# Autodesk Inventor assembly: WheelAssembly3.0
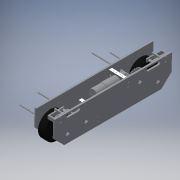
[picture p0: Inventor's stored thumbnail of the model, 180x180]
Saved by Autodesk Inventor 2017 (Build 210142000, 142)
## iProperties
Created: 2017-07-22
Part Number: WheelAssembly3.0
Document SubType Name: Assembly
Designer: User
Author: User
## Documents named in this file (15)
- C:\Robotics\CAD\2017-18_CAD\Miscellaneous\WheelAssembly3.0.iam
- C:\Robotics\CAD\2016-17_CAD\DriveTrain\DriveTrainPlateInside3.0.ipt
- C:\Robotics\CAD\COTSParts\Motors\Andymark 2964  NeveRest 40 Motor.ipt
- C:\Robotics\CAD\COTSParts\Tetrix\tetrix-motor-mounts-1.snapshot.1\Tetrex 2pc motor mount.ipt
- C:\Robotics\CAD\COTSParts\Actobotics\615 parts\615398.25inBoreBeveledGears.ipt
- C:\Robotics\CAD\2016-17_CAD\Custom COTS\4inax.ipt
- C:\Robotics\CAD\COTSParts\Actobotics\615 parts\615106Sprocket.5inBore.25inPitch24Teeth.ipt
- C:\Robotics\CAD\COTSParts\Actobotics\545 parts\545556SetScrewHub.77inPattern.ipt
- C:\Robotics\CAD\COTSParts\Actobotics\615 parts\615114Sprocket.5inBore.25inPitch32Teeth.ipt
- C:\Robotics\CAD\2016-17_CAD\DriveTrain\Tensioner.iam
- C:\Robotics\CAD\COTSParts\Actobotics\545 parts\545456PatternAdapter.77in.625in.ipt
- C:\Robotics\CAD\COTSParts\Wheels\4in Wheel Intergreated Hub 8mm Rev2.ipt
- C:\Robotics\CAD\2016-17_CAD\DriveTrain\MotorFixedPositionMount.ipt
- C:\Robotics\CAD\COTSParts\Actobotics\Thrust Bearings\6655K13.ipt
- C:\Robotics\CAD\2016-17_CAD\DriveTrain\DriveTrainPlateOutside3.0.ipt
## Components (36 placed, 14 different names)
1. DriveTrainPlateInside3.0:1 — Flush:3, Flush:4, Mate:2, Flush:5, Mate:3, Flush:6, Angle:1, Insert:7, Insert:8, Angle:2, Insert:9, Insert:10, Insert:16, Insert:17, Flush:17, Flush:18, Mate:21, Flush:19, Mate:22, Flush:20
2. Andymark 2964  NeveRest 40 Motor:1 — Insert:3, Insert:6, Angle:2
3. Andymark 2964  NeveRest 40 Motor:2 — Insert:4, Insert:5, Angle:1
4. Tetrex 2pc motor mount:1 — Insert:3, Flush:3, Mate:3, Flush:6, Mate:27, Insert:48, Angle:3
5. Tetrex 2pc motor mount:2 — Insert:4, Flush:4, Mate:2, Flush:5, Insert:30, Angle:4
6. 615398.25inBoreBeveledGears:1 — Insert:5, Insert:44
7. 615398.25inBoreBeveledGears:2 — Insert:6, Insert:47
8. 615398.25inBoreBeveledGears:3 — Insert:7, Insert:36
9. 615398.25inBoreBeveledGears:4 — Insert:8, Insert:38
10. 4inax:1 — Insert:9, Mate:18
11. 4inax:2 — Insert:10, Mate:19, Mate:23, Mate:26
12. 615106Sprocket.5inBore.25inPitch24Teeth:2 — Insert:26, Flush:21
13. 4inax:3 — Insert:16
14. 4inax:4 — Insert:17, Mate:14, Mate:25
15. 545556SetScrewHub.77inPattern:3 — Insert:26, Mate:14
16. 615114Sprocket.5inBore.25inPitch32Teeth:2 — Insert:37, Flush:21
17. 545556SetScrewHub.77inPattern:4 — Insert:36, Insert:37, Insert:43
18. Tensioner:1 [sub-assembly] — Flush:17, Flush:18, Mate:21
19. 545556SetScrewHub.77inPattern:5 — Mate:23, Insert:40
20. 545456PatternAdapter.77in.625in:1 — Insert:40, Insert:41
21. 4in Wheel Intergreated Hub 8mm Rev2:1 — Insert:41, Insert:50
22. Tensioner:2 [sub-assembly] — Flush:19, Mate:22, Flush:20
23. 545556SetScrewHub.77inPattern:6 — Insert:27
24. 545456PatternAdapter.77in.625in:2 — Insert:27, Insert:28
25. 4in Wheel Intergreated Hub 8mm Rev2:2 — Insert:28, Insert:49
26. MotorFixedPositionMount:1 — Insert:30, Angle:4
27. MotorFixedPositionMount:2 — Insert:48, Angle:3
28. 545556SetScrewHub.77inPattern:7 — Mate:18, Insert:38, Insert:39, Insert:42
29. 545556SetScrewHub.77inPattern:8 — Insert:35, Mate:19
30. 615114Sprocket.5inBore.25inPitch32Teeth:3 — Insert:39, Flush:22
31. 615106Sprocket.5inBore.25inPitch24Teeth:3 — Insert:35, Flush:22
32. 6655K13:1 — Insert:42
33. 6655K13:2 — Insert:43
34. 6655K13:3 — Insert:44
35. DriveTrainPlateOutside3.0:1 — Mate:25, Mate:26, Mate:27, Insert:49, Insert:50
36. 6655K13:4 — Insert:47
## Relationships (53: Insert 28, Mate 11, Flush 10, Angle 4)
- Insert:3: Andymark 2964  NeveRest 40 Motor:1 ↔ Tetrex 2pc motor mount:1
- Insert:4: Andymark 2964  NeveRest 40 Motor:2 ↔ Tetrex 2pc motor mount:2
- Flush:3 (159.5374 mm): DriveTrainPlateInside3.0:1 ↔ Tetrex 2pc motor mount:1
- Flush:4 (159.5374 mm): DriveTrainPlateInside3.0:1 ↔ Tetrex 2pc motor mount:2
- Insert:5: Andymark 2964  NeveRest 40 Motor:2 ↔ 615398.25inBoreBeveledGears:1
- Mate:2: DriveTrainPlateInside3.0:1 ↔ Tetrex 2pc motor mount:2
- Flush:5 (7.3152 mm): DriveTrainPlateInside3.0:1 ↔ Tetrex 2pc motor mount:2
- Mate:3: DriveTrainPlateInside3.0:1 ↔ Tetrex 2pc motor mount:1
- Flush:6 (-20.3454 mm): DriveTrainPlateInside3.0:1 ↔ Tetrex 2pc motor mount:1
- Angle:1 (0 deg): DriveTrainPlateInside3.0:1 ↔ Andymark 2964  NeveRest 40 Motor:2
- Insert:6: Andymark 2964  NeveRest 40 Motor:1 ↔ 615398.25inBoreBeveledGears:2
- Insert:7 (25.4508 mm): DriveTrainPlateInside3.0:1 ↔ 615398.25inBoreBeveledGears:3
- Insert:8 (25.4508 mm): DriveTrainPlateInside3.0:1 ↔ 615398.25inBoreBeveledGears:4
- Angle:2 (180 deg): DriveTrainPlateInside3.0:1 ↔ Andymark 2964  NeveRest 40 Motor:1
- Insert:9 (-6.35 mm): DriveTrainPlateInside3.0:1 ↔ 4inax:1
- Insert:10 (-6.35 mm): DriveTrainPlateInside3.0:1 ↔ 4inax:2
- Insert:16 (-6.35 mm): DriveTrainPlateInside3.0:1 ↔ 4inax:3
- Insert:17 (-6.35 mm): DriveTrainPlateInside3.0:1 ↔ 4inax:4
- Insert:26: 615106Sprocket.5inBore.25inPitch24Teeth:2 ↔ 545556SetScrewHub.77inPattern:3
- Mate:14: 4inax:4 ↔ 545556SetScrewHub.77inPattern:3
- Insert:27: 545556SetScrewHub.77inPattern:6 ↔ 545456PatternAdapter.77in.625in:2
- Insert:28: 545456PatternAdapter.77in.625in:2 ↔ 4in Wheel Intergreated Hub 8mm Rev2:2
- Insert:30: Tetrex 2pc motor mount:2 ↔ MotorFixedPositionMount:1
- Insert:35: 545556SetScrewHub.77inPattern:8 ↔ 615106Sprocket.5inBore.25inPitch24Teeth:3
- Mate:18: 4inax:1 ↔ 545556SetScrewHub.77inPattern:7
- Mate:19: 4inax:2 ↔ 545556SetScrewHub.77inPattern:8
- Flush:17: DriveTrainPlateInside3.0:1 ↔ Tensioner:1
- Flush:18 (34.925 mm): DriveTrainPlateInside3.0:1 ↔ Tensioner:1
- Mate:21: DriveTrainPlateInside3.0:1 ↔ Tensioner:1
- Flush:19: DriveTrainPlateInside3.0:1 ↔ Tensioner:2
- Mate:22: DriveTrainPlateInside3.0:1 ↔ Tensioner:2
- Flush:20 (-34.925 mm): DriveTrainPlateInside3.0:1 ↔ Tensioner:2
- Insert:36: 615398.25inBoreBeveledGears:3 ↔ 545556SetScrewHub.77inPattern:4
- Insert:37: 615114Sprocket.5inBore.25inPitch32Teeth:2 ↔ 545556SetScrewHub.77inPattern:4
- Flush:21: 615106Sprocket.5inBore.25inPitch24Teeth:2 ↔ 615114Sprocket.5inBore.25inPitch32Teeth:2
- Insert:38: 615398.25inBoreBeveledGears:4 ↔ 545556SetScrewHub.77inPattern:7
- Insert:39: 545556SetScrewHub.77inPattern:7 ↔ 615114Sprocket.5inBore.25inPitch32Teeth:3
- Flush:22: 615114Sprocket.5inBore.25inPitch32Teeth:3 ↔ 615106Sprocket.5inBore.25inPitch24Teeth:3
- Mate:23: 4inax:2 ↔ 545556SetScrewHub.77inPattern:5
- Insert:40: 545556SetScrewHub.77inPattern:5 ↔ 545456PatternAdapter.77in.625in:1
- Insert:41: 545456PatternAdapter.77in.625in:1 ↔ 4in Wheel Intergreated Hub 8mm Rev2:1
- Insert:42: 545556SetScrewHub.77inPattern:7 ↔ 6655K13:1
- Insert:43: 545556SetScrewHub.77inPattern:4 ↔ 6655K13:2
- Insert:44: 615398.25inBoreBeveledGears:1 ↔ 6655K13:3
- Mate:25: 4inax:4 ↔ DriveTrainPlateOutside3.0:1
- Mate:26: 4inax:2 ↔ DriveTrainPlateOutside3.0:1
- Mate:27: Tetrex 2pc motor mount:1 ↔ DriveTrainPlateOutside3.0:1
- Insert:47: 615398.25inBoreBeveledGears:2 ↔ 6655K13:4
- Insert:48: Tetrex 2pc motor mount:1 ↔ MotorFixedPositionMount:2
- Angle:3 (0 deg): Tetrex 2pc motor mount:1 ↔ MotorFixedPositionMount:2
- Angle:4 (0 deg): Tetrex 2pc motor mount:2 ↔ MotorFixedPositionMount:1
- Insert:49 (3.175 mm): 4in Wheel Intergreated Hub 8mm Rev2:2 ↔ DriveTrainPlateOutside3.0:1
- Insert:50 (3.175 mm): 4in Wheel Intergreated Hub 8mm Rev2:1 ↔ DriveTrainPlateOutside3.0:1
